# Autodesk Inventor assembly: 1x1
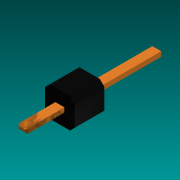
[picture p0: Inventor's stored thumbnail of the model, 180x180]
Saved by Autodesk Inventor 2015 (Build 190159000, 159)
## iProperties
Created: 2014-07-19
Part Number: 1x1
Document SubType Name: Assembly
Designer: Sawaiz Syed
Author: Sawaiz Syed
## Documents named in this file (3)
- E:\Sawaiz\3D Modeling\Projects\Radiation Dector\2.54 Breakaway\1x1.iam
- E:\Sawaiz\3D Modeling\Projects\Radiation Dector\2.54 Breakaway\Holder.ipt
- E:\Sawaiz\3D Modeling\Projects\Radiation Dector\2.54 Breakaway\Pin.ipt
## Components (2 placed, 2 different names)
1. Holder:1 — Mate:1, Mate:2, Flush:1
2. Pin:1 — Mate:1, Mate:2, Flush:1
## Relationships (3: Mate 2, Flush 1)
- Mate:1: Holder:1 ↔ Pin:1
- Mate:2: Holder:1 ↔ Pin:1
- Flush:1 (-5.84 mm): Holder:1 ↔ Pin:1
